# Autodesk Inventor assembly: manual shifter and A bot gearbox_MIR
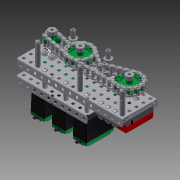
[picture p0: Inventor's stored thumbnail of the model, 180x180]
Saved by Autodesk Inventor 2014 SP1 (Build 180222100, 222)
## iProperties
Created: 2013-08-29
Part Number: manual shifter and A bot gearbox_MIR
Document SubType Name: Assembly
Designer: Ryan
Sending System: SolidWorks 2013
Last Author: Ryan
Author: Ryan
## Documents named in this file (3)
- C:\Users\Ryan\Desktop\pack and go\Workspaces\Workspace\toss up 1st A bot\inventor drive\manual shifter and A bot gearbox_MIR.iam
- C:\Users\Ryan\Desktop\pack and go\Workspaces\Workspace\toss up 1st A bot\inventor drive\manual shifter_MIR.iam
- C:\Users\Ryan\Desktop\pack and go\Workspaces\Workspace\toss up 1st A bot\inventor drive\toss up A bot gearbox_MIR.iam
## Components (2 placed, 2 different names)
1. manual shifter_MIR:1 [sub-assembly] — Mate:1, Flush:1, Flush:2
2. toss up A bot gearbox_MIR:1 [sub-assembly] — Mate:1, Flush:1, Flush:2
## Relationships (3: Flush 2, Mate 1)
- Mate:1: manual shifter_MIR:1 ↔ toss up A bot gearbox_MIR:1
- Flush:1: manual shifter_MIR:1 ↔ toss up A bot gearbox_MIR:1
- Flush:2: manual shifter_MIR:1 ↔ toss up A bot gearbox_MIR:1
